# Autodesk Inventor assembly: side with gearbox_MIR5
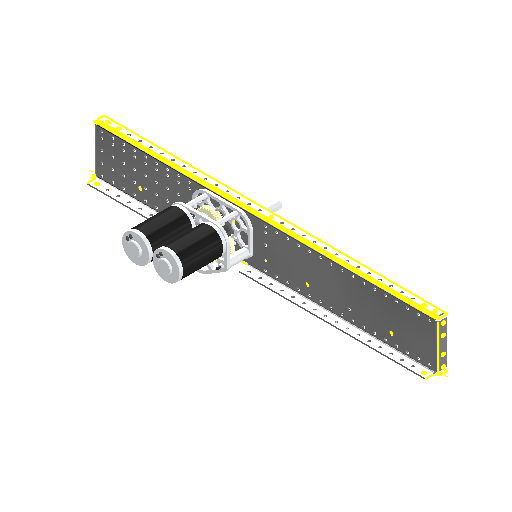
[picture p0: Inventor's stored thumbnail of the model, 512x512]
Saved by Autodesk Inventor 2022 (Build 260153000, 153)
## iProperties
Created: 2022-01-17
Part Number: side with gearbox_MIR5
Document SubType Name: Assembly
Designer: 5126_Cad_5
Author: 5126_Cad_2
## Documents named in this file (3)
- A:\new 2022 cad\new 2022 cad\side with gearbox_MIR5.iam
- A:\new 2022 cad\new 2022 cad\side pannel inner 2 00003_MIR1.ipt
- A:\new 2022 cad\new 2022 cad\WCP DS - Dual Speed Base Kit (217-3423)_MIR5.ipt
## Components (2 placed, 2 different names)
1. side pannel inner 2 00003_MIR1:1 — Mate:3, Mate:2, Mate:1
2. WCP DS - Dual Speed Base Kit (217-3423)_MIR5:1 — Mate:3, Mate:2, Mate:1
## Relationships (3: Mate 3)
- Mate:3: side pannel inner 2 00003_MIR1:1 ↔ WCP DS - Dual Speed Base Kit (217-3423)_MIR5:1
- Mate:2: side pannel inner 2 00003_MIR1:1 ↔ WCP DS - Dual Speed Base Kit (217-3423)_MIR5:1
- Mate:1: side pannel inner 2 00003_MIR1:1 ↔ WCP DS - Dual Speed Base Kit (217-3423)_MIR5:1
